# Autodesk Inventor assembly: Ball_25mm Red
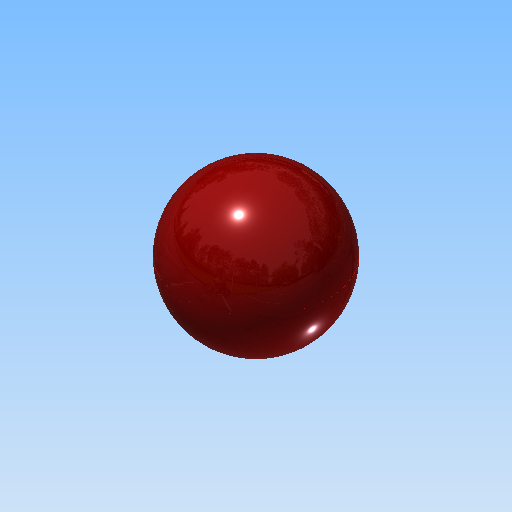
[picture p0: Inventor's stored thumbnail of the model, 512x512]
Saved by Autodesk Inventor 2018.1 (Build 221171000, 171)
## iProperties
Created: 2019-03-22
Part Number: Ball_25mm Red
Document SubType Name: Assembly
Designer: James
Author: James
## Documents named in this file (3)
- C:\Users\admin\Desktop\Ball-Machine\Balls\Ball_25mm Red.iam
- C:\Users\admin\Desktop\Ball-Machine\Balls\Ball_Half Sphere 1.ipt
- C:\Users\admin\Desktop\Ball-Machine\Balls\Steel Ball 25mm.ipt
## Components (3 placed, 2 different names)
1. Ball_Half Sphere 1:1 — Flush:1, Flush:2, Flush:3, Tangent:1, Mate:1, Mate:2
2. Steel Ball 25mm:1 — Tangent:1
3. Ball_Half Sphere 1:2 — Mate:1, Mate:2
## Relationships (6: Flush 3, Mate 2, Tangent 1)
- Flush:1: Ball_Half Sphere 1:1
- Flush:2: Ball_Half Sphere 1:1
- Flush:3: Ball_Half Sphere 1:1
- Tangent:1 (-0.5 mm): Ball_Half Sphere 1:1 ↔ Steel Ball 25mm:1
- Mate:1: Ball_Half Sphere 1:1 ↔ Ball_Half Sphere 1:2
- Mate:2: Ball_Half Sphere 1:1 ↔ Ball_Half Sphere 1:2
